# Autodesk Inventor assembly: cover
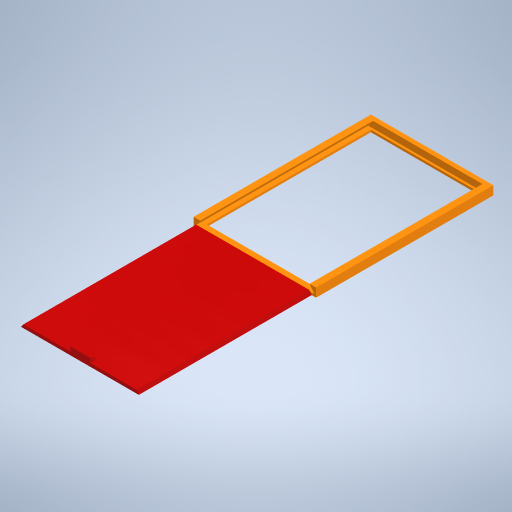
[picture p0: Inventor's stored thumbnail of the model, 512x512]
Saved by Autodesk Inventor 2023 (Build 270158000, 158)
## iProperties
Created: 2023-03-10
Part Number: cover
Document SubType Name: Assembly
Designer: Josh
Author: Josh
## Documents named in this file (3)
- C:\Users\Josh\Documents\HaierFollower\Printed-Upgrades-for-Mingda-Magician-3D-Printers\Protective cover for the screen\SlidingCover\cover.iam
- C:\Users\Josh\Documents\HaierFollower\Printed-Upgrades-for-Mingda-Magician-3D-Printers\Protective cover for the screen\SlidingCover\cover.ipt
- C:\Users\Josh\Documents\HaierFollower\Printed-Upgrades-for-Mingda-Magician-3D-Printers\Protective cover for the screen\SlidingCover\cover2.ipt
## Components (2 placed, 2 different names)
1. cover:1 — Совмещение:1, Заподлицо:1, Совмещение:2, Заподлицо:2, Совмещение:3, Совмещение:4
2. cover2:1 — Совмещение:1, Совмещение:3, Совмещение:4
## Relationships (6: Mate 4, Flush 2)
- Совмещение:1 [Mate]: cover:1 ↔ cover2:1
- Заподлицо:1 [Flush]: cover:1
- Совмещение:2 [Mate]: cover:1
- Заподлицо:2 [Flush]: cover:1
- Совмещение:3 [Mate]: cover:1 ↔ cover2:1
- Совмещение:4 [Mate]: cover:1 ↔ cover2:1
